# Autodesk Inventor assembly: face
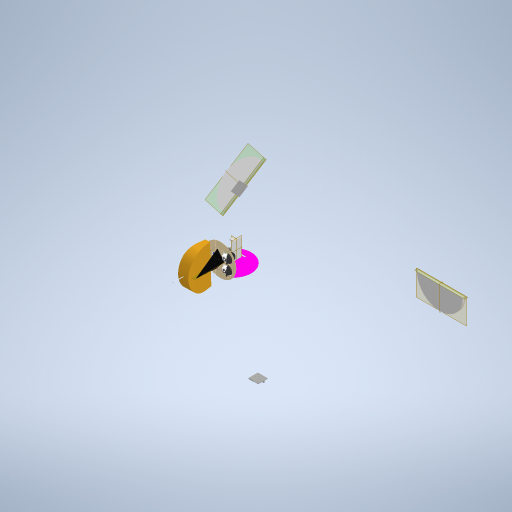
[picture p0: Inventor's stored thumbnail of the model, 512x512]
Saved by Autodesk Inventor 2023.2 (Build 272271030, 271C)
## iProperties
Created: 2024-01-26
Part Number: face
Document SubType Name: Assembly
Designer: I9232
Author: I9232
## Documents named in this file (23)
- D:\!project\fox_n_crow_construction\crow\face\face.iam
- D:\!project\fox_n_crow_construction\crow\face\Сборка глаза вороны.iam
- D:\!project\fox_n_crow_construction\crow\face\Деталь1.ipt
- D:\!project\fox_n_crow_construction\crow\face\Платформа для крыльев лево.ipt
- D:\!project\fox_n_crow_construction\crow\face\Платформа для крыльев право.ipt
- D:\!project\fox_n_crow_construction\crow\face\Сыр.ipt
- D:\!project\fox_n_crow_construction\crow\face\Веер.ipt
- D:\!project\fox_n_crow_construction\crow\face\боковые стороны головы.ipt
- D:\!project\fox_n_crow_construction\crow\face\servoDS3115mg.iam
- D:\!project\fox_n_crow_construction\crow\face\SERVO ARM HORN 25T ALUMINIUM\SERVO ARM HORN 25T ALUMINIUM.ipt
- D:\!project\fox_n_crow_construction\crow\face\Крепление рычага к лицу.ipt
- D:\!project\fox_n_crow_construction\crow\face\Лицо низ.ipt
- D:\!project\fox_n_crow_construction\crow\face\Лицо верх.ipt
- D:\!project\fox_n_crow_construction\crow\face\door_hinge.iam
- D:\!project\fox_n_crow_construction\crow\face\Шапка для головы вороны.ipt
- D:\!project\fox_n_crow_construction\crow\face\Крепление стрелялки.ipt
- D:\!project\fox_n_crow_construction\crow\cheese_shooter\Сборка стрелялки\Сборка стрелялки.iam
- D:\!project\fox_n_crow_construction\crow\face\клюв.ipt
- D:\!project\fox_n_crow_construction\crow\face\крепежная деталь для клюва.ipt
- D:\!project\fox_n_crow_construction\crow\face\Рычаг.ipt
- D:\!project\fox_n_crow_construction\crow\face\door_hinge_MIR.iam
- D:\!project\fox_n_crow_construction\crow\face\боковые стороны головы_MIR3.ipt
- D:\!project\fox_n_crow_construction\crow\face\Нижняя часть головы.ipt
## Components (25 placed, 22 different names)
1. Сборка глаза вороны:1 [sub-assembly] — Заподлицо:1, Совмещение:39
2. Платформа глаз — Заподлицо:1, Заподлицо:4, Заподлицо:5, Заподлицо:6, Совмещение:27, Совмещение:28, Заподлицо:7, Заподлицо:8, Совмещение:38, Совмещение:39, Цилиндрический:9, Совмещение:53
3. Платформа для крыльев лево:1
4. Платформа для крыльев право:1 — Жесткий:1
5. Сыр:1
6. Веер:1 — Жесткий:1
7. Веер:2
8. боковые стороны головы:1 — Совмещение:40, Совмещение:64, Совмещение:65, Совмещение:67
9. servoDS3115mg:1 [sub-assembly] — Цилиндрический:10, Совмещение:40, Совмещение:43, Совмещение:64, Совмещение:65
10. SERVO ARM HORN 25T ALUMINIUM:1 — Цилиндрический:10, Совмещение:43, Цилиндрический:12, Совмещение:59
11. Лицо низ:1 — Угол:2, Цилиндрический:6, Совмещение:19, Совмещение:54, Совмещение:56, Совмещение:57, Совмещение:58, Совмещение:62, Совмещение:63, Цилиндрический:14
12. Лицо верх:1 — Заподлицо:4, Заподлицо:5, Заподлицо:6, Угол:2, Совмещение:30, Совмещение:31, Совмещение:34, Совмещение:51, Цилиндрический:13, Совмещение:66
13. door_hinge:1 [sub-assembly] — Цилиндрический:6, Совмещение:19, Совмещение:38, Цилиндрический:9
14. Шапка для головы вороны:1 — Совмещение:30
15. Крепление стрелялки:1 — Совмещение:27, Совмещение:28, Совмещение:32
16. Сборка стрелялки:1 [sub-assembly] — Заподлицо:7, Совмещение:31, Совмещение:32
17. клюв:2 — Совмещение:34, Заподлицо:8, Заподлицо:9, Совмещение:52
18. Крепление рычага к лицу:1 — Совмещение:56, Совмещение:57, Совмещение:58, Цилиндрический:11
19. крепежная деталь для клюва:1 — Совмещение:54, Совмещение:60, Совмещение:61, Совмещение:62, Совмещение:63
20. крепежная деталь для клюва:2 — Совмещение:51, Заподлицо:9, Совмещение:52
21. Рычаг:1 — Цилиндрический:11, Цилиндрический:12, Совмещение:59
22. клюв:3 — Совмещение:53, Совмещение:60, Совмещение:61
23. door_hinge_MIR:1 [sub-assembly] — Цилиндрический:13, Совмещение:66, Цилиндрический:14
24. боковые стороны головы_MIR3:1
25. Нижняя часть головы:1 — Совмещение:67
## Relationships (43: Mate 27, Flush 7, CylindricalJoint 7, WeldJoint 1, Angle 1)
- Заподлицо:1 [Flush]: Сборка глаза вороны:1 ↔ Платформа глаз
- Жесткий:1 [WeldJoint]: Платформа для крыльев право:1 ↔ Веер:1
- Заподлицо:4 [Flush]: Платформа глаз ↔ Лицо верх:1
- Заподлицо:5 [Flush]: Платформа глаз ↔ Лицо верх:1
- Заподлицо:6 [Flush]: Платформа глаз ↔ Лицо верх:1
- Угол:2 [Angle] (0 deg): Лицо низ:1 ↔ Лицо верх:1
- Цилиндрический:6 [CylindricalJoint]: Лицо низ:1 ↔ door_hinge:1
- Совмещение:19 [Mate]: Лицо низ:1 ↔ door_hinge:1
- Совмещение:27 [Mate]: Платформа глаз ↔ Крепление стрелялки:1
- Совмещение:28 [Mate]: Платформа глаз ↔ Крепление стрелялки:1
- Совмещение:30 [Mate]: Лицо верх:1 ↔ Шапка для головы вороны:1
- Заподлицо:7 [Flush]: Платформа глаз ↔ Сборка стрелялки:1
- Совмещение:31 [Mate]: Лицо верх:1 ↔ Сборка стрелялки:1
- Совмещение:32 [Mate]: Крепление стрелялки:1 ↔ Сборка стрелялки:1
- Совмещение:34 [Mate]: Лицо верх:1 ↔ клюв:2
- Заподлицо:8 [Flush]: Платформа глаз ↔ клюв:2
- Совмещение:38 [Mate]: Платформа глаз ↔ door_hinge:1
- Совмещение:39 [Mate]: Сборка глаза вороны:1 ↔ Платформа глаз
- Цилиндрический:9 [CylindricalJoint]: Платформа глаз ↔ door_hinge:1
- Цилиндрический:10 [CylindricalJoint]: servoDS3115mg:1 ↔ SERVO ARM HORN 25T ALUMINIUM:1
- Совмещение:40 [Mate]: боковые стороны головы:1 ↔ servoDS3115mg:1
- Совмещение:43 [Mate]: servoDS3115mg:1 ↔ SERVO ARM HORN 25T ALUMINIUM:1
- Совмещение:51 [Mate]: Лицо верх:1 ↔ крепежная деталь для клюва:2
- Заподлицо:9 [Flush]: клюв:2 ↔ крепежная деталь для клюва:2
- Совмещение:52 [Mate]: клюв:2 ↔ крепежная деталь для клюва:2
- Совмещение:53 [Mate]: Платформа глаз ↔ клюв:3
- Совмещение:54 [Mate]: Лицо низ:1 ↔ крепежная деталь для клюва:1
- Совмещение:56 [Mate]: Лицо низ:1 ↔ Крепление рычага к лицу:1
- Совмещение:57 [Mate]: Лицо низ:1 ↔ Крепление рычага к лицу:1
- Совмещение:58 [Mate]: Лицо низ:1 ↔ Крепление рычага к лицу:1
- Цилиндрический:11 [CylindricalJoint]: Крепление рычага к лицу:1 ↔ Рычаг:1
- Цилиндрический:12 [CylindricalJoint]: SERVO ARM HORN 25T ALUMINIUM:1 ↔ Рычаг:1
- Совмещение:59 [Mate]: SERVO ARM HORN 25T ALUMINIUM:1 ↔ Рычаг:1
- Совмещение:60 [Mate]: крепежная деталь для клюва:1 ↔ клюв:3
- Совмещение:61 [Mate]: крепежная деталь для клюва:1 ↔ клюв:3
- Совмещение:62 [Mate]: Лицо низ:1 ↔ крепежная деталь для клюва:1
- Совмещение:63 [Mate]: Лицо низ:1 ↔ крепежная деталь для клюва:1
- Совмещение:64 [Mate]: боковые стороны головы:1 ↔ servoDS3115mg:1
- Совмещение:65 [Mate]: боковые стороны головы:1 ↔ servoDS3115mg:1
- Цилиндрический:13 [CylindricalJoint]: Лицо верх:1 ↔ door_hinge_MIR:1
- Совмещение:66 [Mate]: Лицо верх:1 ↔ door_hinge_MIR:1
- Цилиндрический:14 [CylindricalJoint]: Лицо низ:1 ↔ door_hinge_MIR:1
- Совмещение:67 [Mate]: боковые стороны головы:1 ↔ Нижняя часть головы:1
